# Autodesk Inventor assembly: assemble
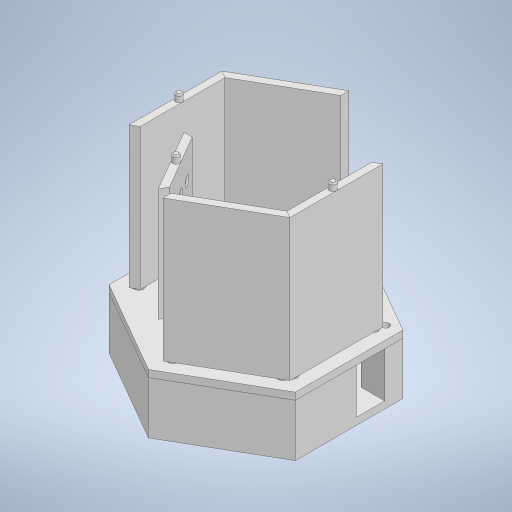
[picture p0: Inventor's stored thumbnail of the model, 512x512]
Saved by Autodesk Inventor 2024 (Build 280153000, 153)
## iProperties
Created: 2024-03-18
Part Number: assemble
Document SubType Name: Assembly
Designer: SSAFY
Author: SSAFY
## Documents named in this file (8)
- C:\Users\SSAFY\Desktop\TIL\3D\3D\2nd\assemble.iam
- C:\Users\SSAFY\Desktop\TIL\3D\3D\2nd\pi_case_bottom.ipt
- C:\Users\SSAFY\Desktop\TIL\3D\3D\2nd\pi_case_top.ipt
- C:\Users\SSAFY\Desktop\TIL\3D\3D\2nd\col.ipt
- C:\Users\SSAFY\Desktop\TIL\3D\3D\2nd\col_MIR.ipt
- C:\Users\SSAFY\Desktop\TIL\3D\3D\2nd\col_MIR1.ipt
- C:\Users\SSAFY\Desktop\TIL\3D\3D\2nd\inner_case_bottom.ipt
- C:\Users\SSAFY\Desktop\TIL\3D\3D\2nd\col_face.ipt
## Components (8 placed, 7 different names)
1. pi_case_bottom:2 — 플러쉬:1, 플러쉬:2, 플러쉬:3, 메이트:1, 메이트:2, 메이트:4
2. pi_case_top:2 — 메이트:1, 메이트:2, 메이트:4, 메이트:5, 메이트:6, 메이트:7, 메이트:9, 메이트:10, 메이트:11, 메이트:13
3. col:1 — 메이트:5, 메이트:6, 메이트:7
4. col:2 — 메이트:9, 메이트:10, 메이트:11
5. col_MIR:1
6. col_MIR1:1
7. inner_case_bottom:1 — 메이트:13, 메이트:14, 메이트:15, 메이트:16
8. col_face:1 — 메이트:15, 메이트:16
## Relationships (16: Mate 13, Flush 3)
- 플러쉬:1 [Flush]: pi_case_bottom:2
- 플러쉬:2 [Flush]: pi_case_bottom:2
- 플러쉬:3 [Flush]: pi_case_bottom:2
- 메이트:1 [Mate]: pi_case_bottom:2 ↔ pi_case_top:2
- 메이트:2 [Mate]: pi_case_bottom:2 ↔ pi_case_top:2
- 메이트:4 [Mate]: pi_case_bottom:2 ↔ pi_case_top:2
- 메이트:5 [Mate]: pi_case_top:2 ↔ col:1
- 메이트:6 [Mate]: pi_case_top:2 ↔ col:1
- 메이트:7 [Mate]: pi_case_top:2 ↔ col:1
- 메이트:9 [Mate]: pi_case_top:2 ↔ col:2
- 메이트:10 [Mate]: pi_case_top:2 ↔ col:2
- 메이트:11 [Mate]: pi_case_top:2 ↔ col:2
- 메이트:13 [Mate] (4 mm): pi_case_top:2 ↔ inner_case_bottom:1
- 메이트:14 [Mate]: inner_case_bottom:1
- 메이트:15 [Mate]: inner_case_bottom:1 ↔ col_face:1
- 메이트:16 [Mate]: inner_case_bottom:1 ↔ col_face:1
